# Autodesk Inventor assembly: Electronica
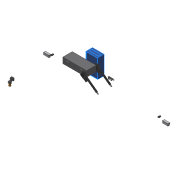
[picture p0: Inventor's stored thumbnail of the model, 180x180]
Saved by Autodesk Inventor 2020 (Build 240168000, 168)
## iProperties
Created: 2020-02-27
Part Number: Electronica
Document SubType Name: Assembly
Designer: Juan Carlos Botero
Author: Juan Carlos Botero
## Documents named in this file (12)
- D:\Drives\OneDrive\Carlos_2\02 TRABAJOS\MULTIPLO\Conveyor\ORIGINAL_RUA\Electronica.iam
- D:\Drives\OneDrive\Carlos_2\02 TRABAJOS\MULTIPLO\Conveyor\ORIGINAL_RUA\Botón de emergencia _1_.iam
- D:\Drives\OneDrive\Carlos_2\02 TRABAJOS\MULTIPLO\Conveyor\ORIGINAL_RUA\Botón de emergencia _2_.iam
- D:\Drives\OneDrive\Carlos_2\02 TRABAJOS\MULTIPLO\Conveyor\ORIGINAL_RUA\Luz _1_.iam
- D:\Drives\OneDrive\Carlos_2\02 TRABAJOS\MULTIPLO\Conveyor\ORIGINAL_RUA\Beacon _1_.iam
- D:\Drives\OneDrive\Carlos_2\02 TRABAJOS\MULTIPLO\Conveyor\ORIGINAL_RUA\Actuador lineal pequeño _1_.iam
- D:\Drives\OneDrive\Carlos_2\02 TRABAJOS\MULTIPLO\Conveyor\ORIGINAL_RUA\Bateria LiFePo4 51 (1).iam
- D:\Drives\OneDrive\Carlos_2\02 TRABAJOS\MULTIPLO\Conveyor\ORIGINAL_RUA\caja electrica _1_.iam
- D:\Drives\OneDrive\Carlos_2\02 TRABAJOS\MULTIPLO\Conveyor\ORIGINAL_RUA\Actuador lineal _2_.iam
- D:\Drives\OneDrive\Carlos_2\02 TRABAJOS\MULTIPLO\Conveyor\ORIGINAL_RUA\Actuador lineal _1_.iam
- D:\Drives\OneDrive\Carlos_2\02 TRABAJOS\MULTIPLO\Conveyor\ORIGINAL_RUA\Botonera 3 botones _2_.iam
- D:\Drives\OneDrive\Carlos_2\02 TRABAJOS\MULTIPLO\Conveyor\ORIGINAL_RUA\Botonera 3 botones _2__1.iam
## Components (11 placed, 10 different names)
1. Botón de emergencia <1>:1 [sub-assembly]
2. Botón de emergencia <2>:1 [sub-assembly]
3. Luz <1>:1 [sub-assembly]
4. Beacon <1>:1 [sub-assembly]
5. Actuador lineal pequeño <1>:1 [sub-assembly]
6. Bateria LiFePo4 51 (1):1 [sub-assembly] — Flush:1
7. caja electrica <1>:1 [sub-assembly] — Flush:1
8. Actuador lineal <2>:1 [sub-assembly]
9. Actuador lineal <1>:1 [sub-assembly]
10. Botonera 3 botones <2>:1 [sub-assembly]
11. Botonera 3 botones <2>:2 [sub-assembly]
## Relationships (1: Flush 1)
- Flush:1 (-50 mm): Bateria LiFePo4 51 (1):1 ↔ caja electrica <1>:1
